# Autodesk Inventor assembly: A6M60-400H2B1-M17
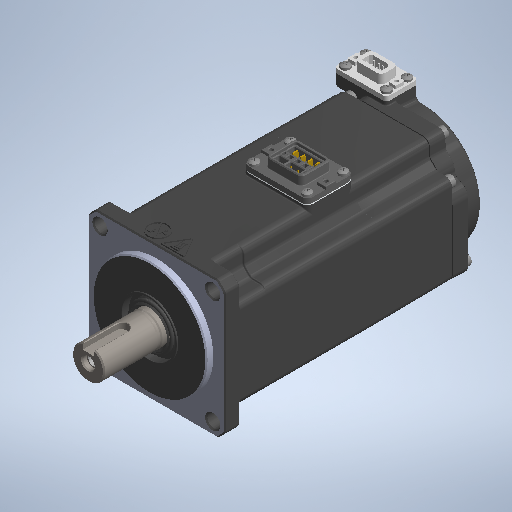
[picture p0: Inventor's stored thumbnail of the model, 512x512]
Saved by Autodesk Inventor 2025.3 (Build 293356000, 356)
## iProperties
Created: 2024-09-06
Part Number: A6M60-400H2B1-M17
Description: STEP AP214
Document SubType Name: Assembly
Designer: louis
Mass: 2432.92 g
Surface Area: 700.755 cm^2
Volume: 310.206 cm^3
Density: 7.84291 g/cm^3
Sending System: SolidWorks 2020
Preprocessor: SwSTEP 2.0
Title: 60-400W-ÓÐÓÍ·âÓÐÖÆ¶¯Æ÷(RSK1-H060A04B30E).STEP
## Documents named in this file (12)
- C:\Users\louis\OneDrive\Desktop\R_Trident\02_CAD\01_Standard_Parts\A6M60-400H2B1-M17\A6M60-400H2B1-M17.iam
- C:\Users\louis\OneDrive\Desktop\R_Trident\02_CAD\01_Standard_Parts\A6M60-400H2B1-M17\2142000001_»ú¿ÇÃ«Å÷_RSK1-H060A04B30S36.ipt
- C:\Users\louis\OneDrive\Desktop\R_Trident\02_CAD\01_Standard_Parts\A6M60-400H2B1-M17\2174000002_ºó¶Ë¸ÇÃ«Å÷_RSK1-H060A04B30E36.ipt
- C:\Users\louis\OneDrive\Desktop\R_Trident\02_CAD\01_Standard_Parts\A6M60-400H2B1-M17\2181000001_ºó¸Ç_RSK1-H060A04B30S36.ipt
- C:\Users\louis\OneDrive\Desktop\R_Trident\02_CAD\01_Standard_Parts\A6M60-400H2B1-M17\3231000003_¹´°åÂÝË¿ÐÍ6pinÁ¬½ÓÆ÷²å×ù_GAMC3063.ipt
- C:\Users\louis\OneDrive\Desktop\R_Trident\02_CAD\01_Standard_Parts\A6M60-400H2B1-M17\Ð¡µç»ú±àÂë¶Ë×Ó.ipt
- C:\Users\louis\OneDrive\Desktop\R_Trident\02_CAD\01_Standard_Parts\A6M60-400H2B1-M17\60·¨À¼Öá.ipt
- C:\Users\louis\OneDrive\Desktop\R_Trident\02_CAD\01_Standard_Parts\A6M60-400H2B1-M17\3220000001_ÓÍ·â_TC15x25x4(NBR).ipt
- C:\Users\louis\OneDrive\Desktop\R_Trident\02_CAD\01_Standard_Parts\A6M60-400H2B1-M17\3130000001_Æ½¼ü_B5x5x14(GBT1096-2003 ´øÆð¼üÂÝ¿×M3).ipt
- C:\Users\louis\OneDrive\Desktop\R_Trident\02_CAD\01_Standard_Parts\A6M60-400H2B1-M17\3111000001_ÄÚÁù½ÇÔ²ÖùÍ·ÂÝ¶¤_M2.5x10(GBT70.1-2000 Ð¿ÄøºÏ½ð ºÚÉ« ÄÍÂä 12.9¼¶£©.ipt
- C:\Users\louis\OneDrive\Desktop\R_Trident\02_CAD\01_Standard_Parts\A6M60-400H2B1-M17\3114000001_Ê®×Ö²ÛÅÌÍ·×Ô¼·ÂÝ¶¤_M2x5(GBT6560-2014 Ð¿ÄøºÏ½ð ºÚÉ«).ipt
- C:\Users\louis\OneDrive\Desktop\R_Trident\02_CAD\01_Standard_Parts\A6M60-400H2B1-M17\3111000002_ÄÚÁù½ÇÔ²ÖùÍ·ÂÝ¶¤_M2.5x40(GBT70.1-2000 Ð¿ÄøºÏ½ð ºÚÉ« ÄÍÂä 12.9¼¶£©.ipt
## Components (24 placed, 24 different names)
1. 2142000001_»ú¿ÇÃ«Å÷_RSK1-H060A04B30S36_1 — Flush:1, Mate:1
2. 2174000002_ºó¶Ë¸ÇÃ«Å÷_RSK1-H060A04B30E36_2
3. 2181000001_ºó¸Ç_RSK1-H060A04B30S36_3
4. 3231000003_¹´°åÂÝË¿ÐÍ6pinÁ¬½ÓÆ÷²å×ù_GAMC3063_4
5. Ð¡µç»ú±àÂë¶Ë×Ó_5
6. 60·¨À¼Öá_6 — Flush:1, Flush:2, Mate:1, Mate:2, Mate:3
7. 3220000001_ÓÍ·â_TC15x25x4(NBR)_7
8. 3130000001_Æ½¼ü_B5x5x14(GBT1096-2003 ´øÆð¼üÂÝ¿×M3)_8 — Flush:2, Mate:2, Mate:3
9. 3111000001_ÄÚÁù½ÇÔ²ÖùÍ·ÂÝ¶¤_M2.5x10(GBT70.1-2000 Ð¿ÄøºÏ½ð ºÚÉ« ÄÍÂä 12.9¼¶£©_9
10. 3114000001_Ê®×Ö²ÛÅÌÍ·×Ô¼·ÂÝ¶¤_M2x5(GBT6560-2014 Ð¿ÄøºÏ½ð ºÚÉ«)_10
11. 3114000001_Ê®×Ö²ÛÅÌÍ·×Ô¼·ÂÝ¶¤_M2x5(GBT6560-2014 Ð¿ÄøºÏ½ð ºÚÉ«)_11
12. 3114000001_Ê®×Ö²ÛÅÌÍ·×Ô¼·ÂÝ¶¤_M2x5(GBT6560-2014 Ð¿ÄøºÏ½ð ºÚÉ«)_12
13. 3114000001_Ê®×Ö²ÛÅÌÍ·×Ô¼·ÂÝ¶¤_M2x5(GBT6560-2014 Ð¿ÄøºÏ½ð ºÚÉ«)_13
14. 3114000001_Ê®×Ö²ÛÅÌÍ·×Ô¼·ÂÝ¶¤_M2x5(GBT6560-2014 Ð¿ÄøºÏ½ð ºÚÉ«)_14
15. 3114000001_Ê®×Ö²ÛÅÌÍ·×Ô¼·ÂÝ¶¤_M2x5(GBT6560-2014 Ð¿ÄøºÏ½ð ºÚÉ«)_15
16. 3114000001_Ê®×Ö²ÛÅÌÍ·×Ô¼·ÂÝ¶¤_M2x5(GBT6560-2014 Ð¿ÄøºÏ½ð ºÚÉ«)_16
17. 3114000001_Ê®×Ö²ÛÅÌÍ·×Ô¼·ÂÝ¶¤_M2x5(GBT6560-2014 Ð¿ÄøºÏ½ð ºÚÉ«)_17
18. 3111000001_ÄÚÁù½ÇÔ²ÖùÍ·ÂÝ¶¤_M2.5x10(GBT70.1-2000 Ð¿ÄøºÏ½ð ºÚÉ« ÄÍÂä 12.9¼¶£©_18
19. 3111000001_ÄÚÁù½ÇÔ²ÖùÍ·ÂÝ¶¤_M2.5x10(GBT70.1-2000 Ð¿ÄøºÏ½ð ºÚÉ« ÄÍÂä 12.9¼¶£©_19
20. 3111000001_ÄÚÁù½ÇÔ²ÖùÍ·ÂÝ¶¤_M2.5x10(GBT70.1-2000 Ð¿ÄøºÏ½ð ºÚÉ« ÄÍÂä 12.9¼¶£©_20
21. 3111000002_ÄÚÁù½ÇÔ²ÖùÍ·ÂÝ¶¤_M2.5x40(GBT70.1-2000 Ð¿ÄøºÏ½ð ºÚÉ« ÄÍÂä 12.9¼¶£©_21
22. 3111000002_ÄÚÁù½ÇÔ²ÖùÍ·ÂÝ¶¤_M2.5x40(GBT70.1-2000 Ð¿ÄøºÏ½ð ºÚÉ« ÄÍÂä 12.9¼¶£©_22
23. 3111000002_ÄÚÁù½ÇÔ²ÖùÍ·ÂÝ¶¤_M2.5x40(GBT70.1-2000 Ð¿ÄøºÏ½ð ºÚÉ« ÄÍÂä 12.9¼¶£©_23
24. 3111000002_ÄÚÁù½ÇÔ²ÖùÍ·ÂÝ¶¤_M2.5x40(GBT70.1-2000 Ð¿ÄøºÏ½ð ºÚÉ« ÄÍÂä 12.9¼¶£©_24
## Relationships (5: Mate 3, Flush 2)
- Flush:1 (-30 mm): 2142000001_»ú¿ÇÃ«Å÷_RSK1-H060A04B30S36_1 ↔ 60·¨À¼Öá_6
- Flush:2: 60·¨À¼Öá_6 ↔ 3130000001_Æ½¼ü_B5x5x14(GBT1096-2003 ´øÆð¼üÂÝ¿×M3)_8
- Mate:1: 2142000001_»ú¿ÇÃ«Å÷_RSK1-H060A04B30S36_1 ↔ 60·¨À¼Öá_6
- Mate:2: 60·¨À¼Öá_6 ↔ 3130000001_Æ½¼ü_B5x5x14(GBT1096-2003 ´øÆð¼üÂÝ¿×M3)_8
- Mate:3: 60·¨À¼Öá_6 ↔ 3130000001_Æ½¼ü_B5x5x14(GBT1096-2003 ´øÆð¼üÂÝ¿×M3)_8
